# Autodesk Inventor assembly: weight_holder
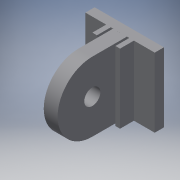
[picture p0: Inventor's stored thumbnail of the model, 180x180]
Saved by Autodesk Inventor 2016 (Build 200138000, 138)
## iProperties
Created: 2016-08-02
Part Number: weight_holder
Document SubType Name: Assembly
Designer: ajar021
Author: ajar021
## Documents named in this file (3)
- C:\Users\ajar021\Documents\weight_holder.iam
- C:\Users\ajar021\Documents\weight_holder_base.ipt
- C:\Users\ajar021\Documents\weight_holder_string_loop.ipt
## Components (2 placed, 2 different names)
1. weight_holder_base:1 — Flush:1
2. weight_holder_string_loop:1 — Flush:1
## Relationships (1: Flush 1)
- Flush:1: weight_holder_base:1 ↔ weight_holder_string_loop:1
